# Autodesk Inventor assembly: Assembly1
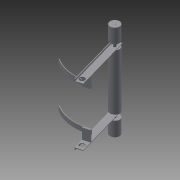
[picture p0: Inventor's stored thumbnail of the model, 180x180]
Saved by Autodesk Inventor 2015 (Build 190159000, 159)
## iProperties
Created: 2016-01-20
Part Number: Assembly1
Document SubType Name: Assembly
Designer: 278648
Author: 278648
## Documents named in this file (7)
- C:\Users\278648\Documents\CADstuff\Assembly1.iam
- C:\Users\278648\Documents\CADstuff\arm.ipt
- C:\Users\278648\Documents\CADstuff\rail.ipt
- C:\Users\278648\Documents\CADstuff\axel.ipt
- C:\Users\278648\Documents\CADstuff\Part8.ipt
- C:\Users\278648\Documents\CADstuff\Part9.ipt
- C:\Users\278648\Documents\CADstuff\Part10.ipt
## Components (10 placed, 6 different names)
1. arm:1 — Flush:1, Mate:1, Flush:2, Mate:3, Mate:21, Flush:11
2. arm:2 — Flush:1, Mate:1, Flush:2, Mate:4, Mate:6, Mate:15, Mate:27, Flush:10
3. rail:1 — Mate:3, Mate:5, Flush:7, Mate:29
4. axel:1 — Mate:13, Mate:14, Mate:23, Mate:24, Flush:8, Mate:25, Mate:26, Flush:9
5. rail:2 — Mate:4, Mate:5, Mate:6, Flush:5, Flush:6, Mate:20
6. Part8:1 — Mate:13, Mate:14, Mate:15
7. Part9:1 — Flush:5, Flush:6, Mate:20, Flush:10
8. Part9:2 — Mate:21, Flush:7, Mate:29, Flush:11
9. Part10:1 — Mate:23, Mate:24, Flush:8
10. Part10:2 — Mate:25, Mate:26, Flush:9, Mate:27
## Relationships (25: Mate 16, Flush 9)
- Flush:1: arm:1 ↔ arm:2
- Mate:1 (304.8 mm): arm:1 ↔ arm:2
- Flush:2: arm:1 ↔ arm:2
- Mate:3: arm:1 ↔ rail:1
- Mate:4: arm:2 ↔ rail:2
- Mate:5 (190.5 mm): rail:1 ↔ rail:2
- Mate:6 (31.75 mm): arm:2 ↔ rail:2
- Mate:13: axel:1 ↔ Part8:1
- Mate:14: axel:1 ↔ Part8:1
- Mate:15 (3.175 mm): arm:2 ↔ Part8:1
- Flush:5: rail:2 ↔ Part9:1
- Flush:6: rail:2 ↔ Part9:1
- Mate:20: rail:2 ↔ Part9:1
- Mate:21: arm:1 ↔ Part9:2
- Flush:7: rail:1 ↔ Part9:2
- Mate:23: axel:1 ↔ Part10:1
- Mate:24: axel:1 ↔ Part10:1
- Flush:8: axel:1 ↔ Part10:1
- Mate:25: axel:1 ↔ Part10:2
- Mate:26: axel:1 ↔ Part10:2
- Flush:9: axel:1 ↔ Part10:2
- Mate:27 (12.7 mm): arm:2 ↔ Part10:2
- Mate:29: rail:1 ↔ Part9:2
- Flush:10: arm:2 ↔ Part9:1
- Flush:11: arm:1 ↔ Part9:2
